# Autodesk Inventor assembly: X Axis
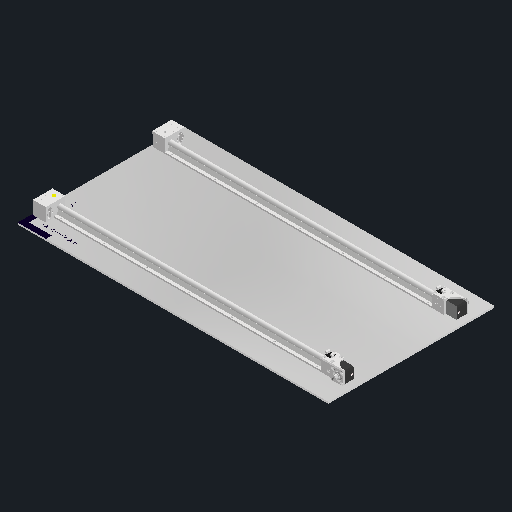
[picture p0: Inventor's stored thumbnail of the model, 512x512]
Saved by Autodesk Inventor 2026 (Build 300175000, 175)
## iProperties
Created: 2024-11-25
Part Number: X Axis
Document SubType Name: Assembly
Designer: jerem
Author: jerem
## Documents named in this file (7)
- C:\Users\jerem\Documents\GitHub\Perovskite-Automated-Synthesis-System\CAD\Gantry\X Axis\X Axis.iam
- C:\Users\jerem\Documents\GitHub\Perovskite-Automated-Synthesis-System\CAD\Non 3D Printed Parts\Base Plate.ipt
- C:\Users\jerem\Documents\GitHub\Perovskite-Automated-Synthesis-System\CAD\Non 3D Printed Parts\Linear Rails\Linear Rail.ipt
- C:\Users\jerem\Documents\GitHub\Perovskite-Automated-Synthesis-System\CAD\Gantry\X Axis\X Axis Motor End.iam
- C:\Users\jerem\Documents\GitHub\Perovskite-Automated-Synthesis-System\CAD\Gantry\X Axis\Belt Tensioner End.iam
- C:\Users\jerem\Documents\GitHub\Perovskite-Automated-Synthesis-System\CAD\Gantry\X Axis\X Axis Motor End_MIR.iam
- C:\Users\jerem\Documents\GitHub\Perovskite-Automated-Synthesis-System\CAD\Gantry\X Axis\Belt Tensioner End_MIR.iam
## Components (7 placed, 6 different names)
1. Base Plate:1 — Flush:1, Flush:2, Mate:14, Mate:17, Mate:28, Mate:32
2. Linear Rail:1 — Flush:1, Mate:3, Mate:18, Mate:26, Flush:2, Mate:30, Mate:31
3. Linear Rail:2 — Mate:3, Mate:15, Mate:16, Mate:27, Mate:29
4. X Axis Motor End:1 [sub-assembly] — Mate:14, Mate:15, Mate:16
5. Belt Tensioner End:1 [sub-assembly] — Mate:17, Mate:18, Mate:26
6. Belt Tensioner End_MIR:1 [sub-assembly] — Mate:27, Mate:28, Mate:29
7. X Axis Motor End_MIR:1 [sub-assembly] — Mate:30, Mate:31, Mate:32
## Relationships (18: Mate 15, Flush 3)
- Flush:1 (20 mm): Base Plate:1 ↔ Linear Rail:1
- Flush:2 (78 mm): Base Plate:1 ↔ Linear Rail:1
- [Mate]: Base Plate:1 ↔ Linear Rail:1
- [Mate]: Base Plate:1 ↔ Linear Rail:2
- [Flush]: Linear Rail:1 ↔ Linear Rail:2
- Mate:3 (350 mm): Linear Rail:1 ↔ Linear Rail:2
- Mate:14: Base Plate:1 ↔ X Axis Motor End:1
- Mate:15: Linear Rail:2 ↔ X Axis Motor End:1
- Mate:16: Linear Rail:2 ↔ X Axis Motor End:1
- Mate:17: Base Plate:1 ↔ Belt Tensioner End:1
- Mate:18: Linear Rail:1 ↔ Belt Tensioner End:1
- Mate:26: Linear Rail:1 ↔ Belt Tensioner End:1
- Mate:27: Linear Rail:2 ↔ Belt Tensioner End_MIR:1
- Mate:28: Base Plate:1 ↔ Belt Tensioner End_MIR:1
- Mate:29: Linear Rail:2 ↔ Belt Tensioner End_MIR:1
- Mate:30: Linear Rail:1 ↔ X Axis Motor End_MIR:1
- Mate:31: Linear Rail:1 ↔ X Axis Motor End_MIR:1
- Mate:32: Base Plate:1 ↔ X Axis Motor End_MIR:1
